# Autodesk Inventor assembly: saucerAssembly2
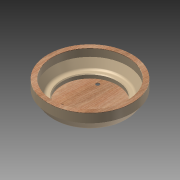
[picture p0: Inventor's stored thumbnail of the model, 180x180]
Saved by Autodesk Inventor 2015 SP1 (Build 190203100, 203)
## iProperties
Created: 2015-02-16
Part Number: saucerAssembly2
Document SubType Name: Assembly
Designer: Jostein
Author: Jostein
## Documents named in this file (5)
- C:\Users\Jostein\Desktop\Saucer\saucerAssembly2.iam
- C:\Users\Jostein\Desktop\Saucer\bottom.ipt
- C:\Users\Jostein\Desktop\Saucer\body.ipt
- C:\Users\Jostein\Desktop\Saucer\top.ipt
- C:\Users\Jostein\Desktop\Saucer\coating.ipt
## Components (4 placed, 4 different names)
1. bottom:1
2. body:1 — Flush:1, Flush:2, Flush:3
3. top:1 — Flush:2, Flush:3
4. coating:1 — Flush:4
## Relationships (4: Flush 4)
- Flush:1: body:1
- Flush:2: body:1 ↔ top:1
- Flush:3: body:1 ↔ top:1
- Flush:4: coating:1
